# Autodesk Inventor assembly: Programmer_mini
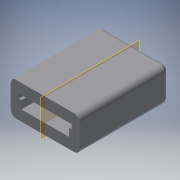
[picture p0: Inventor's stored thumbnail of the model, 180x180]
Saved by Autodesk Inventor 2018 (Build 220112000, 112)
## iProperties
Created: 2018-05-15
Part Number: Programmer_mini
Document SubType Name: Assembly
Designer: Mandus
Author: Mandus
## Documents named in this file (3)
- C:\Users\Mandus\Dropbox\Skola\Projekt\Kretsn_Brillz_V2\3D\Programmer_mini\Programmer_mini.iam
- C:\Users\Mandus\Dropbox\Skola\Projekt\Kretsn_Brillz_V2\3D\Programmer_mini\Top.ipt
- C:\Users\Mandus\Dropbox\Skola\Projekt\Kretsn_Brillz_V2\3D\Programmer_mini\Bottom.ipt
## Components (2 placed, 2 different names)
1. Top:1 — Flush:2, Flush:3, Mate:1
2. Bottom:1 — Flush:2, Flush:3, Mate:1
## Relationships (3: Flush 2, Mate 1)
- Flush:2: Top:1 ↔ Bottom:1
- Flush:3 (3 mm): Top:1 ↔ Bottom:1
- Mate:1 (1.7 mm): Top:1 ↔ Bottom:1
